# Autodesk Inventor assembly: motor_case
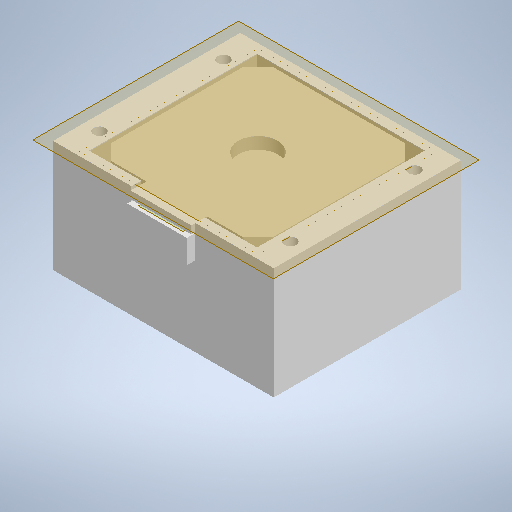
[picture p0: Inventor's stored thumbnail of the model, 512x512]
Saved by Autodesk Inventor 2025.2 (Build 292293000, 293)
## iProperties
Created: 2024-11-24
Part Number: motor_case
Document SubType Name: Assembly
Designer: dell
Author: dell
## Documents named in this file (3)
- D:\兵庫県立大\creap\motor_case.iam
- D:\兵庫県立大\creap\stepper_motor.ipt
- D:\兵庫県立大\creap\motor_case2.ipt
## Components (2 placed, 2 different names)
1. stepper_motor:1 — リジッド:1
2. motor_case2:1 — リジッド:1
## Relationships (1: WeldJoint 1)
- リジッド:1 [WeldJoint]: stepper_motor:1 ↔ motor_case2:1
